# Autodesk Inventor assembly: wormgear_pol_base
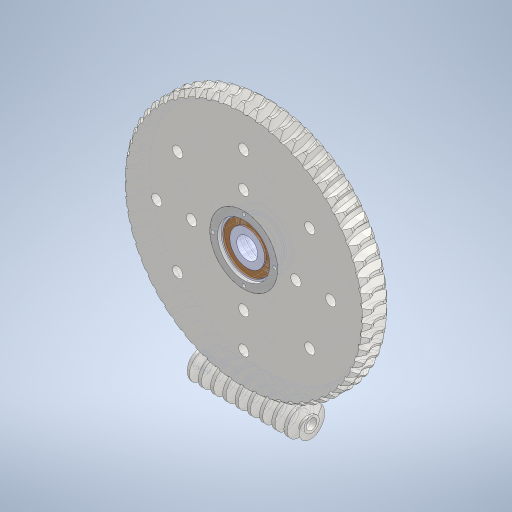
[picture p0: Inventor's stored thumbnail of the model, 512x512]
Saved by Autodesk Inventor 2024 (Build 280153000, 153)
## iProperties
Created: 2025-12-08
Part Number: wormgear_pol_base
Document SubType Name: Assembly
Designer: schar
Author: schar
## Documents named in this file (4)
- C:\Users\schar\Desktop\projectBlueprint\AMSTS\hardware\wormgear_pol_base.iam
- C:\Users\schar\Desktop\projectBlueprint\AMSTS\hardware\Assembly1\Design Accelerator\Worm Gears3.iam
- C:\Users\schar\Desktop\projectBlueprint\AMSTS\hardware\base_bearing_holder.ipt
- C:\Users\schar\Desktop\projectBlueprint\AMSTS\hardware\ROLAMENTO 6201RS 32X12.ipt
## Components (3 placed, 3 different names)
1. Worm Gears:5 [sub-assembly] — Mate:1, Mate:2
2. base_bearing_holder:1 — Mate:2, Mate:3
3. ROLAMENTO 6201RS 32X12:1 — Mate:1, Mate:3
## Relationships (3: Mate 3)
- Mate:1: Worm Gears:5 ↔ ROLAMENTO 6201RS 32X12:1
- Mate:2: Worm Gears:5 ↔ base_bearing_holder:1
- Mate:3: base_bearing_holder:1 ↔ ROLAMENTO 6201RS 32X12:1
